# Autodesk Inventor assembly: ASY DMF filter package v2.1
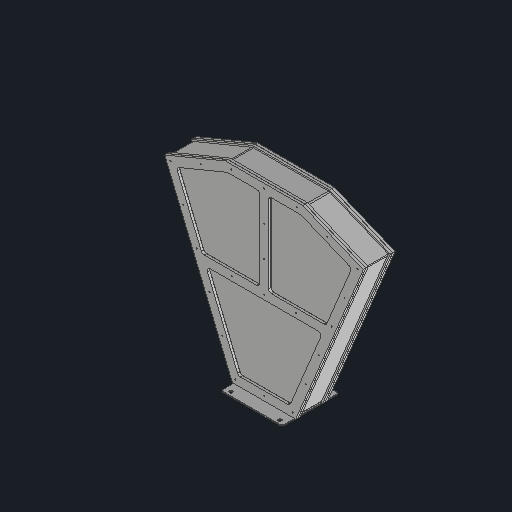
[picture p0: Inventor's stored thumbnail of the model, 512x512]
Saved by Autodesk Inventor 2026.2 (Build 302298000, 298)
## iProperties
Created: 2024-05-16
Part Number: ASY DMF filter package v2.1
Document SubType Name: Assembly
Designer: admin
Author: admin
## Documents named in this file (17)
- C:\Users\admin\Documents\Inventor\DMF-Disk-Micro-Filter\Барабан v2.1\ASY DMF filter package v2.1.iam
- C:\Users\admin\Documents\Inventor\DMF-Disk-Micro-Filter\Барабан v2.1\DMF 01 51 outside frame v2.1.ipt
- ДМС 201 Внешняя рамка.ipt
- C:\Users\admin\Documents\Inventor\DMF-Disk-Micro-Filter\Барабан v2.1\DMF 01 52 Top sheet v2.1.ipt
- C:\Users\admin\Documents\Inventor\DMF-Disk-Micro-Filter\Барабан v2.1\DMF 01 53 side part v2.1.ipt
- C:\Users\admin\Documents\Inventor\DMF-Disk-Micro-Filter\Барабан v2.1\DMF 01 54 lower sheet v2.1.ipt
- C:\Users\admin\Documents\Inventor\DMF-Disk-Micro-Filter\Барабан v2.1\DMF 01 56 Крепление сетки к кассете v2.1.ipt
- ДМС 206 Крепление сетки к кассете.ipt
- C:\Users\admin\Documents\Inventor\DMF-Disk-Micro-Filter\Барабан v2.1\DMF 01 57 Сетка кассеты v2.1.ipt
- ДМС 207 Сетка кассеты.ipt
- C:\Users\admin\Documents\Inventor\DMF-Disk-Micro-Filter\Барабан v2.1\DMF 01 51 outside frame_MIR1 v2.1.ipt
- C:\Users\admin\Documents\Inventor\DMF-Disk-Micro-Filter\Барабан v2.1\DMF 01 56 Крепление сетки к кассете_MIR1 v2.1.ipt
- C:\Users\admin\Documents\Inventor\DMF-Disk-Micro-Filter\Барабан v2.1\DMF 01 57 Сетка кассеты_MIR1 v2.1.ipt
- C:\Users\admin\Documents\Inventor\DMF-Disk-Micro-Filter\Барабан v2.1\DMF 2.1 01 42 Gear way 2.ipt
- C:\Users\admin\Documents\Inventor\DMF-Disk-Micro-Filter\ContentCenter\en-US\DIN EN 24 017\ISO 4017 - M10 x 35DIN EN.ipt
- C:\Users\admin\Documents\Inventor\DMF-Disk-Micro-Filter\ContentCenter\en-US\ISO 4032(1)\ISO 4032 - M10DIN EN.ipt
- C:\Users\admin\Documents\Inventor\DMF-Disk-Micro-Filter\ContentCenter\en-US\ISO 4032(1)\ISO 4032 - M8DIN EN.ipt
## Components (16 placed, 13 different names)
1. DMF 01 51 outside frame v2.1.ipt:1 — Rigid:8
2. DMF 01 52 Top sheet v2.1.ipt:1 — Rigid:7
3. DMF 01 53 side part v2.1.ipt:1
4. DMF 01 54 lower sheet v2.1.ipt:1 — Rigid:8, Rigid:9, Rotational:3, Rotational:4
5. DMF 01 56 Крепление сетки к кассете v2.1.ipt:1
6. DMF 01 57 Сетка кассеты v2.1.ipt:1
7. DMF 01 53 side part v2.1.ipt:2
8. DMF 01 51 outside frame_MIR1 v2.1.ipt:1 — Rigid:7
9. DMF 01 56 Крепление сетки к кассете_MIR1 v2.1.ipt:1
10. DMF 01 57 Сетка кассеты_MIR1 v2.1.ipt:1
11. DMF 2.1 01 42 Gear way 2.ipt:1 — Mate:4, Mate:5, Rigid:9, Mate:6, Mate:8, Insert:5
12. DIN EN 24017 M10 x 35:2 — Rotational:3, Mate:7
13. DIN EN 24017 M10 x 35:1 — Rotational:4
14. DIN EN 24032 M10:1 — Mate:7, Mate:8
15. DIN EN 24032 M10:2
16. DIN EN 24032 M8:5 — Insert:5
## Relationships (21: WeldJoint 8, Mate 7, RevoluteJoint 4, Insert 2)
- [WeldJoint]: DMF 01 51 outside frame v2.1.ipt:1 ↔ DMF 01 57 Сетка кассеты v2.1.ipt:1
- [WeldJoint]: DMF 01 51 outside frame v2.1.ipt:1 ↔ DMF 01 52 Top sheet v2.1.ipt:1
- [RevoluteJoint]: DMF 01 51 outside frame v2.1.ipt:1 ↔ DMF 01 53 side part v2.1.ipt:1
- [Mate]: DMF 01 51 outside frame v2.1.ipt:1 ↔ DMF 01 53 side part v2.1.ipt:1
- [WeldJoint] (0.5 mm): DMF 01 51 outside frame v2.1.ipt:1 ↔ DMF 01 56 Крепление сетки к кассете v2.1.ipt:1
- [RevoluteJoint]: DMF 01 51 outside frame v2.1.ipt:1 ↔ DMF 01 53 side part v2.1.ipt:2
- [Mate]: DMF 01 51 outside frame v2.1.ipt:1 ↔ DMF 01 53 side part v2.1.ipt:2
- [WeldJoint] (0.5 mm): DMF 01 51 outside frame_MIR1 v2.1.ipt:1 ↔ DMF 01 56 Крепление сетки к кассете_MIR1 v2.1.ipt:1
- [WeldJoint]: DMF 01 51 outside frame_MIR1 v2.1.ipt:1 ↔ DMF 01 57 Сетка кассеты_MIR1 v2.1.ipt:1
- Rigid:7 [WeldJoint]: DMF 01 52 Top sheet v2.1.ipt:1 ↔ DMF 01 51 outside frame_MIR1 v2.1.ipt:1
- Rigid:8 [WeldJoint]: DMF 01 51 outside frame v2.1.ipt:1 ↔ DMF 01 54 lower sheet v2.1.ipt:1
- Mate:4: DMF 2.1 01 42 Gear way 2.ipt:1
- Mate:5: DMF 2.1 01 42 Gear way 2.ipt:1
- Rigid:9 [WeldJoint] (5 mm): DMF 01 54 lower sheet v2.1.ipt:1 ↔ DMF 2.1 01 42 Gear way 2.ipt:1
- Mate:6: DMF 2.1 01 42 Gear way 2.ipt:1
- Rotational:3 [RevoluteJoint]: DMF 01 54 lower sheet v2.1.ipt:1 ↔ DIN EN 24017 M10 x 35:2
- Rotational:4 [RevoluteJoint]: DMF 01 54 lower sheet v2.1.ipt:1 ↔ DIN EN 24017 M10 x 35:1
- Mate:7: DIN EN 24017 M10 x 35:2 ↔ DIN EN 24032 M10:1
- Mate:8: DMF 2.1 01 42 Gear way 2.ipt:1 ↔ DIN EN 24032 M10:1
- [Insert]: DMF 2.1 01 42 Gear way 2.ipt:1 ↔ DIN EN 24032 M10:2
- Insert:5: DMF 2.1 01 42 Gear way 2.ipt:1 ↔ DIN EN 24032 M8:5
## Named parameters: d0_d1 = 0 mm, d1_d3 = 0 mm, d2_d4 = 0 mm, d3_d5 = 90 deg, d4_d6 = 0 mm, d5_d7 = 0.5 mm, d6_d8 = 0 mm, d7_d9 = -90 deg, d8_d10 = 0 mm
